# Autodesk Inventor assembly: 足回り
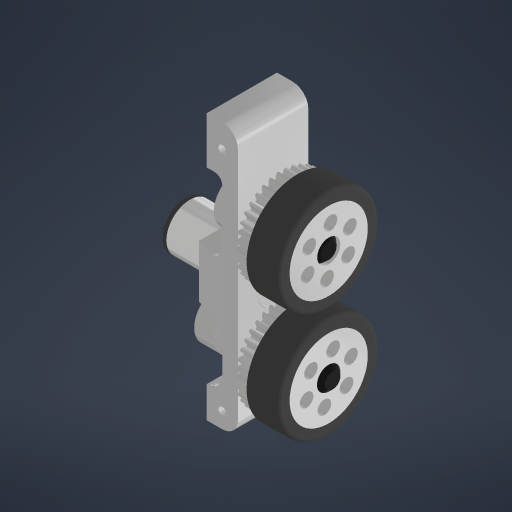
[picture p0: Inventor's stored thumbnail of the model, 512x512]
Saved by Autodesk Inventor 2023 (Build 270158000, 158)
## iProperties
Created: 2022-03-31
Part Number: 足回り
Document SubType Name: Assembly
Designer: neko2
Author: neko2
## Documents named in this file (12)
- C:\Users\neko2\Desktop\SaponseEx\CAD\足回り.iam
- C:\Users\neko2\Desktop\SaponseEx\CAD\MotorMount.ipt
- C:\Users\neko2\Desktop\SaponseEx\CAD\FL673ZZ.ipt
- C:\Users\neko2\Desktop\SaponseEx\CAD\HeikoPin.ipt
- C:\Users\neko2\Desktop\SaponseEx\CAD\RT-PN v2.ipt
- C:\Users\neko2\Desktop\SaponseEx\CAD\Tire.ipt
- C:\Users\neko2\Desktop\SaponseEx\CAD\Stopper.ipt
- C:\Users\neko2\Desktop\SaponseEx\CAD\Magnet.iam
- C:\Users\neko2\Desktop\SaponseEx\CAD\Magnet_Simple.ipt
- C:\Users\neko2\Desktop\SaponseEx\CAD\Magnet.ipt
- C:\Users\neko2\Desktop\SaponseEx\CAD\Gear.iam
- C:\Users\neko2\Desktop\SaponseEx\CAD\CoreLessMotor.ipt
## Components (17 placed, 10 different names)
1. MotorMount:1 — メイト:24, メイト:27, リジッド:21, リジッド:19, リジッド:20, リジッド:23, フラッシュ:29, リジッド:31
2. CoreLessMotor:1 — リジッド:31, 回転:1
3. FL673ZZ:1 — リジッド:20, メイト:29
4. FL673ZZ:2 — リジッド:21, メイト:28, メイト:30
5. FL673ZZ:3 — リジッド:19, 円柱状:22, メイト:33
6. FL673ZZ:4 — リジッド:23, 円柱状:21, メイト:32
7. HeikoPin:1 — 円柱状:17, 円柱状:19, リジッド:28, 円柱状:22
8. HeikoPin:2 — 円柱状:18, 円柱状:20, 円柱状:21, メイト:31
9. RT-PN v2:1 — 回転:1
10. Tire:1 — リジッド:30
11. Tire:2 — リジッド:29
12. Stopper:1 — 円柱状:18, メイト:29
13. Magnet:1 [sub-assembly] — 円柱状:17, メイト:28
14. Magnet_Simple:1 — メイト:30, 円柱状:19, リジッド:27
15. Magnet:2 — リジッド:27
16. Gear:1 [sub-assembly] — 円柱状:20, メイト:31, メイト:32, リジッド:30
17. Gear:2 [sub-assembly] — リジッド:28, メイト:33, リジッド:29
## Relationships (25: WeldJoint 9, Mate 8, CylindricalJoint 6, Flush 1, RevoluteJoint 1)
- メイト:24 [Mate]: MotorMount:1
- メイト:27 [Mate]: MotorMount:1
- 円柱状:17 [CylindricalJoint]: HeikoPin:1 ↔ Magnet:1
- リジッド:21 [WeldJoint]: MotorMount:1 ↔ FL673ZZ:2
- リジッド:19 [WeldJoint]: MotorMount:1 ↔ FL673ZZ:3
- リジッド:20 [WeldJoint]: MotorMount:1 ↔ FL673ZZ:1
- リジッド:23 [WeldJoint]: MotorMount:1 ↔ FL673ZZ:4
- フラッシュ:29 [Flush]: MotorMount:1
- メイト:28 [Mate]: FL673ZZ:2 ↔ Magnet:1
- 円柱状:18 [CylindricalJoint]: HeikoPin:2 ↔ Stopper:1
- メイト:29 [Mate]: FL673ZZ:1 ↔ Stopper:1
- メイト:30 [Mate]: FL673ZZ:2 ↔ Magnet_Simple:1
- 円柱状:19 [CylindricalJoint]: HeikoPin:1 ↔ Magnet_Simple:1
- リジッド:27 [WeldJoint]: Magnet_Simple:1 ↔ Magnet:2
- 円柱状:20 [CylindricalJoint]: HeikoPin:2 ↔ Gear:1
- 円柱状:21 [CylindricalJoint]: FL673ZZ:4 ↔ HeikoPin:2
- メイト:31 [Mate]: HeikoPin:2 ↔ Gear:1
- メイト:32 [Mate]: FL673ZZ:4 ↔ Gear:1
- リジッド:28 [WeldJoint]: HeikoPin:1 ↔ Gear:2
- 円柱状:22 [CylindricalJoint]: FL673ZZ:3 ↔ HeikoPin:1
- メイト:33 [Mate]: FL673ZZ:3 ↔ Gear:2
- リジッド:29 [WeldJoint]: Tire:2 ↔ Gear:2
- リジッド:30 [WeldJoint]: Tire:1 ↔ Gear:1
- リジッド:31 [WeldJoint]: MotorMount:1 ↔ CoreLessMotor:1
- 回転:1 [RevoluteJoint] (0.2 mm): CoreLessMotor:1 ↔ RT-PN v2:1
